# Autodesk Inventor assembly: Socket
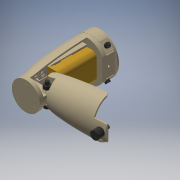
[picture p0: Inventor's stored thumbnail of the model, 180x180]
Saved by Autodesk Inventor 2019.1 (Build 231200000, 200)
## iProperties
Created: 2018-05-25
Part Number: Socket
Material: 一般
Document SubType Name: Assembly
Designer: sktom
Sending System: Autodesk Translation Framework v7.1.0.215
Preprocessor: ST-DEVELOPER v17
Title: D:/Home/Desktop/前腕ユニット_70mm_newJoint v14.step
Author: sktometometo_
## Documents named in this file (16)
- D:\CloudStrage\OneDrive\CADMech\HbSizeSMech\UnitSocket\UnitSocket.iam
- D:\CloudStrage\OneDrive\CADMech\HbSizeSMech\UnitSocket\UnitSocket\S-SO-1.ipt
- D:\CloudStrage\OneDrive\CADMech\HbSizeSMech\UnitSocket\UnitSocket\Parts_CoilSpring_CP_0.5-4.5-6.5.ipt
- D:\CloudStrage\OneDrive\CADMech\HbSizeSMech\UnitSocket\UnitSocket\S-SO-3.ipt
- D:\CloudStrage\OneDrive\CADMech\HbSizeSMech\UnitSocket\UnitSocket\Parts_Screw_M2_L6.ipt
- D:\CloudStrage\OneDrive\CADMech\HbSizeSMech\UnitSocket\UnitSocket\S-SO-2.ipt
- D:\CloudStrage\OneDrive\CADMech\HbSizeSMech\UnitSocket\UnitSocket\S-SO-4.ipt
- D:\CloudStrage\OneDrive\CADMech\HbSizeSMech\UnitSocket\UnitSocket\Parts_Bolt_M4_L25.ipt
- D:\CloudStrage\OneDrive\CADMech\HbSizeSMech\UnitSocket\UnitSocket\Parts_Nuts_M4.ipt
- D:\CloudStrage\OneDrive\CADMech\HbSizeSMech\UnitSocket\UnitSocket\Parts_Bolt_M3_L10.ipt
- D:\CloudStrage\OneDrive\CADMech\HbSizeSMech\UnitSocket\UnitSocket\S-Socket-Template.ipt
- D:\CloudStrage\OneDrive\CADMech\HbSizeSMech\UnitSocket\UnitSocket\Parts_PCB_BatteryProbePCB.ipt
- D:\CloudStrage\OneDrive\CADMech\HbSizeSMech\UnitSocket\UnitSocket\Parts_Probe_101050-003.ipt
- D:\CloudStrage\OneDrive\CADMech\HbSizeSMech\UnitSocket\UnitSocket\Parts_Screw_M2_L4.ipt
- D:\CloudStrage\OneDrive\CADMech\HbSizeSMech\UnitSocket\UnitSocket\Parts_DressBolt_M3_L10.ipt
- D:\CloudStrage\OneDrive\CADMech\HbSizeSMech\UnitSocket\UnitSocket\Parts_Battery_NB-2LH.ipt
## Components (22 placed, 15 different names)
1. S-SO-1:1 — 挿入:1, 挿入:2, 挿入:3, 挿入:10, 挿入:13, 円柱状:1
2. S-SO-2:1 — 挿入:10, 挿入:11, 挿入:12, リジッド:1
3. S-SO-3:1 — 挿入:2, 挿入:3, 挿入:4, 挿入:5, 挿入:6, 挿入:7, 挿入:16, 挿入:17, メイト:1, メイト:2, フラッシュ:1
4. S-SO-4:1 — 挿入:9
5. S-Socket-Template:1 — 挿入:13, 円柱状:1, 挿入:14, 挿入:15, リジッド:2
6. Parts_CoilSpring_CP_0.5-4.5-6.5:1 — 挿入:1, 挿入:9
7. Parts_Screw_M2_L6:1 — 挿入:4
8. Parts_Screw_M2_L6:2 — 挿入:5
9. Parts_Screw_M2_L6:3 — 挿入:7
10. Parts_Screw_M2_L6:4 — 挿入:6
11. Parts_Bolt_M4_L25:1 — 挿入:11
12. Parts_Nuts_M4:1 — 挿入:12
13. Parts_DressBolt_M3_L10:1 — リジッド:1
14. Parts_Bolt_M3_L10:2 — 挿入:14
15. Parts_Bolt_M3_L10:3 — 挿入:15
16. Parts_Bolt_M3_L10:4 — リジッド:2
17. Parts_PCB_BatteryProbePCB:1 — 挿入:16, 挿入:17, 挿入:18, 挿入:19, 挿入:20, 挿入:21
18. Parts_Probe_101050-003:1 — 挿入:18
19. Parts_Probe_101050-003:2 — 挿入:19
20. Parts_Screw_M2_L4:1 — 挿入:20
21. Parts_Screw_M2_L4:2 — 挿入:21
22. Parts_Battery_NB-2LH:1 — メイト:1, メイト:2, フラッシュ:1
## Relationships (26: Insert 20, WeldJoint 2, Mate 2, CylindricalJoint 1, Flush 1)
- 挿入:1 [Insert]: S-SO-1:1 ↔ Parts_CoilSpring_CP_0.5-4.5-6.5:1
- 挿入:2 [Insert]: S-SO-1:1 ↔ S-SO-3:1
- 挿入:3 [Insert]: S-SO-1:1 ↔ S-SO-3:1
- 挿入:4 [Insert]: S-SO-3:1 ↔ Parts_Screw_M2_L6:1
- 挿入:5 [Insert]: S-SO-3:1 ↔ Parts_Screw_M2_L6:2
- 挿入:6 [Insert]: S-SO-3:1 ↔ Parts_Screw_M2_L6:4
- 挿入:7 [Insert]: S-SO-3:1 ↔ Parts_Screw_M2_L6:3
- 挿入:9 [Insert]: S-SO-4:1 ↔ Parts_CoilSpring_CP_0.5-4.5-6.5:1
- 挿入:10 [Insert] (0.5 mm): S-SO-1:1 ↔ S-SO-2:1
- 挿入:11 [Insert]: S-SO-2:1 ↔ Parts_Bolt_M4_L25:1
- 挿入:12 [Insert]: S-SO-2:1 ↔ Parts_Nuts_M4:1
- リジッド:1 [WeldJoint]: S-SO-2:1 ↔ Parts_DressBolt_M3_L10:1
- 挿入:13 [Insert]: S-SO-1:1 ↔ S-Socket-Template:1
- 円柱状:1 [CylindricalJoint]: S-SO-1:1 ↔ S-Socket-Template:1
- 挿入:14 [Insert]: S-Socket-Template:1 ↔ Parts_Bolt_M3_L10:2
- 挿入:15 [Insert]: S-Socket-Template:1 ↔ Parts_Bolt_M3_L10:3
- リジッド:2 [WeldJoint]: S-Socket-Template:1 ↔ Parts_Bolt_M3_L10:4
- 挿入:16 [Insert]: S-SO-3:1 ↔ Parts_PCB_BatteryProbePCB:1
- 挿入:17 [Insert]: S-SO-3:1 ↔ Parts_PCB_BatteryProbePCB:1
- 挿入:18 [Insert]: Parts_PCB_BatteryProbePCB:1 ↔ Parts_Probe_101050-003:1
- 挿入:19 [Insert]: Parts_PCB_BatteryProbePCB:1 ↔ Parts_Probe_101050-003:2
- 挿入:20 [Insert]: Parts_PCB_BatteryProbePCB:1 ↔ Parts_Screw_M2_L4:1
- 挿入:21 [Insert]: Parts_PCB_BatteryProbePCB:1 ↔ Parts_Screw_M2_L4:2
- メイト:1 [Mate]: S-SO-3:1 ↔ Parts_Battery_NB-2LH:1
- メイト:2 [Mate]: S-SO-3:1 ↔ Parts_Battery_NB-2LH:1
- フラッシュ:1 [Flush]: S-SO-3:1 ↔ Parts_Battery_NB-2LH:1
